# Autodesk Inventor assembly: drive with fourbar linkage
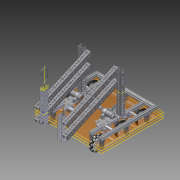
[picture p0: Inventor's stored thumbnail of the model, 180x180]
Saved by Autodesk Inventor 2013 (Build 170138000, 138)
## iProperties
Created: 2013-12-21
Part Number: drive with fourbar linkage
Document SubType Name: Assembly
Designer: kahohbein
Author: kahohbein
## Documents named in this file (12)
- C:\Users\kahohbein\Documents\GitHub\2013-2014_BlockParty\CAD\drive with fourbar linkage.iam
- C:\Users\kahohbein\Documents\GitHub\2013-2014_BlockParty\CAD\Drive\Final Drive Complete\Driveopen2.iam
- C:\Users\kahohbein\Documents\GitHub\2013-2014_BlockParty\CAD\COTSParts\Tetrix\Tetrix flat plate.ipt
- C:\Users\kahohbein\Documents\GitHub\2013-2014_BlockParty\CAD\COTSParts\Tetrix\Tetrix channel 288mm.ipt
- C:\Users\kahohbein\Documents\GitHub\2013-2014_BlockParty\CAD\COTSParts\Tetrix\Tetrix channel 32mm.ipt
- C:\Users\kahohbein\Documents\GitHub\2013-2014_BlockParty\CAD\COTSParts\Tetrix\Tetrix Channel 416mm.ipt
- C:\Users\kahohbein\Documents\GitHub\2013-2014_BlockParty\CAD\COTSParts\Tetrix\Bronze bushing.ipt
- C:\Users\kahohbein\Documents\GitHub\2013-2014_BlockParty\CAD\COTSParts\Tetrix\Tetrix channel 160mm.ipt
- C:\Users\kahohbein\Documents\GitHub\2013-2014_BlockParty\CAD\Tetrix channel 288mm modifyed.ipt
- C:\Users\kahohbein\Documents\GitHub\2013-2014_BlockParty\CAD\Lift\MK3\winch MK3.iam
- C:\Users\kahohbein\Documents\GitHub\2013-2014_BlockParty\CAD\COTSParts\Tetrix\Tetrix motor mount.ipt
- C:\Users\kahohbein\Documents\GitHub\2013-2014_BlockParty\CAD\Lift\MK3\hook prototype.ipt
## Components (29 placed, 11 different names)
1. Driveopen2:1 [sub-assembly] — Mate:1, Mate:2, Mate:3, Mate:4, Mate:5, Mate:6
2. Tetrix flat plate:1 — Mate:2, Mate:3, Mate:4, Mate:8, Mate:9, Mate:15, Mate:16, Mate:65, Mate:66, Mate:70
3. Tetrix flat plate:2 — Mate:1, Mate:5, Mate:6, Mate:7, Mate:10, Mate:11, Mate:12, Mate:67, Mate:68, Mate:69
4. Tetrix channel 288mm:1 — Mate:7, Mate:10, Mate:13, Mate:14, Mate:19, Mate:31, Mate:32, Mate:35, Mate:36, Mate:43, Mate:44, Mate:47, Mate:48
5. Tetrix channel 288mm:2 — Mate:8, Mate:9, Mate:17, Mate:18, Mate:20, Mate:25, Mate:28, Mate:29, Mate:30, Mate:38, Mate:41, Mate:42, Mate:50, Mate:51
6. Tetrix channel 32mm:1 — Mate:15, Mate:16, Mate:17, Mate:18
7. Tetrix channel 32mm:2 — Mate:11, Mate:12, Mate:13, Mate:14
8. Tetrix Channel 416mm:1 — Mate:20, Mate:21, Mate:24, Mate:26, Mate:74, Mate:75
9. Tetrix Channel 416mm:2 — Mate:19, Mate:21, Mate:33, Mate:34, Mate:60, Mate:61
10. Tetrix Channel 416mm:3 — Mate:38, Mate:39, Mate:40, Mate:53, Mate:55, Mate:59
11. Tetrix Channel 416mm:4 — Mate:39, Mate:45, Mate:46, Mate:55, Mate:73
12. Bronze bushing:1 — Mate:24, Mate:26, Mate:27
13. Bronze bushing:2 — Mate:25, Mate:27, Mate:28
14. Bronze bushing:3 — Mate:29, Mate:30
15. Bronze bushing:4 — Mate:31, Mate:36, Mate:37
16. Bronze bushing:5 — Mate:33, Mate:34, Mate:37
17. Bronze bushing:6 — Mate:32, Mate:35
18. Bronze bushing:7 — Mate:41, Mate:51
19. Bronze bushing:8 — Mate:42, Mate:50, Mate:52
20. Bronze bushing:9 — Mate:45, Mate:46, Mate:52
21. Bronze bushing:10 — Mate:40, Mate:53, Mate:54
22. Bronze bushing:11 — Mate:44, Mate:48, Mate:54
23. Bronze bushing:12 — Mate:43, Mate:47
24. Tetrix channel 288mm modifyed:1 — Mate:59, Mate:60, Mate:61, Mate:76, Mate:77, Mate:78
25. winch MK3:1 [sub-assembly] — Mate:71, Mate:72
26. Tetrix motor mount:1 — Mate:65, Mate:66, Mate:70, Mate:71
27. Tetrix motor mount:2 — Mate:67, Mate:68, Mate:69, Mate:72
28. Tetrix channel 160mm:1 — Mate:73, Mate:74, Mate:75
29. hook prototype:1 — Mate:76, Mate:77, Mate:78
## Relationships (69: Mate 69)
- Mate:1: Driveopen2:1 ↔ Tetrix flat plate:2
- Mate:2: Driveopen2:1 ↔ Tetrix flat plate:1
- Mate:3 (139.7 mm): Driveopen2:1 ↔ Tetrix flat plate:1
- Mate:4 (63.5 mm): Driveopen2:1 ↔ Tetrix flat plate:1
- Mate:5 (139.7 mm): Driveopen2:1 ↔ Tetrix flat plate:2
- Mate:6 (63.5 mm): Driveopen2:1 ↔ Tetrix flat plate:2
- Mate:7: Tetrix flat plate:2 ↔ Tetrix channel 288mm:1
- Mate:8: Tetrix flat plate:1 ↔ Tetrix channel 288mm:2
- Mate:9: Tetrix flat plate:1 ↔ Tetrix channel 288mm:2
- Mate:10: Tetrix flat plate:2 ↔ Tetrix channel 288mm:1
- Mate:11: Tetrix flat plate:2 ↔ Tetrix channel 32mm:2
- Mate:12: Tetrix flat plate:2 ↔ Tetrix channel 32mm:2
- Mate:13: Tetrix channel 288mm:1 ↔ Tetrix channel 32mm:2
- Mate:14: Tetrix channel 288mm:1 ↔ Tetrix channel 32mm:2
- Mate:15: Tetrix flat plate:1 ↔ Tetrix channel 32mm:1
- Mate:16: Tetrix flat plate:1 ↔ Tetrix channel 32mm:1
- Mate:17: Tetrix channel 288mm:2 ↔ Tetrix channel 32mm:1
- Mate:18: Tetrix channel 288mm:2 ↔ Tetrix channel 32mm:1
- Mate:19: Tetrix channel 288mm:1 ↔ Tetrix Channel 416mm:2
- Mate:20: Tetrix channel 288mm:2 ↔ Tetrix Channel 416mm:1
- Mate:21: Tetrix Channel 416mm:1 ↔ Tetrix Channel 416mm:2
- Mate:24: Tetrix Channel 416mm:1 ↔ Bronze bushing:1
- Mate:25: Tetrix channel 288mm:2 ↔ Bronze bushing:2
- Mate:26: Tetrix Channel 416mm:1 ↔ Bronze bushing:1
- Mate:27 (6.35 mm): Bronze bushing:1 ↔ Bronze bushing:2
- Mate:28: Tetrix channel 288mm:2 ↔ Bronze bushing:2
- Mate:29: Tetrix channel 288mm:2 ↔ Bronze bushing:3
- Mate:30: Tetrix channel 288mm:2 ↔ Bronze bushing:3
- Mate:31: Tetrix channel 288mm:1 ↔ Bronze bushing:4
- Mate:32: Tetrix channel 288mm:1 ↔ Bronze bushing:6
- Mate:33: Tetrix Channel 416mm:2 ↔ Bronze bushing:5
- Mate:34: Tetrix Channel 416mm:2 ↔ Bronze bushing:5
- Mate:35: Tetrix channel 288mm:1 ↔ Bronze bushing:6
- Mate:36: Tetrix channel 288mm:1 ↔ Bronze bushing:4
- Mate:37 (6.35 mm): Bronze bushing:4 ↔ Bronze bushing:5
- Mate:38: Tetrix channel 288mm:2 ↔ Tetrix Channel 416mm:3
- Mate:39: Tetrix Channel 416mm:3 ↔ Tetrix Channel 416mm:4
- Mate:40: Tetrix Channel 416mm:3 ↔ Bronze bushing:10
- Mate:41: Tetrix channel 288mm:2 ↔ Bronze bushing:7
- Mate:42: Tetrix channel 288mm:2 ↔ Bronze bushing:8
- Mate:43: Tetrix channel 288mm:1 ↔ Bronze bushing:12
- Mate:44: Tetrix channel 288mm:1 ↔ Bronze bushing:11
- Mate:45: Tetrix Channel 416mm:4 ↔ Bronze bushing:9
- Mate:46: Tetrix Channel 416mm:4 ↔ Bronze bushing:9
- Mate:47: Tetrix channel 288mm:1 ↔ Bronze bushing:12
- Mate:48: Tetrix channel 288mm:1 ↔ Bronze bushing:11
- Mate:50: Tetrix channel 288mm:2 ↔ Bronze bushing:8
- Mate:51: Tetrix channel 288mm:2 ↔ Bronze bushing:7
- Mate:52 (6.35 mm): Bronze bushing:8 ↔ Bronze bushing:9
- Mate:53: Tetrix Channel 416mm:3 ↔ Bronze bushing:10
- Mate:54 (6.35 mm): Bronze bushing:10 ↔ Bronze bushing:11
- Mate:55: Tetrix Channel 416mm:3 ↔ Tetrix Channel 416mm:4
- Mate:59: Tetrix Channel 416mm:3 ↔ Tetrix channel 288mm modifyed:1
- Mate:60: Tetrix Channel 416mm:2 ↔ Tetrix channel 288mm modifyed:1
- Mate:61 (3.175 mm): Tetrix Channel 416mm:2 ↔ Tetrix channel 288mm modifyed:1
- Mate:65: Tetrix flat plate:1 ↔ Tetrix motor mount:1
- Mate:66: Tetrix flat plate:1 ↔ Tetrix motor mount:1
- Mate:67: Tetrix flat plate:2 ↔ Tetrix motor mount:2
- Mate:68: Tetrix flat plate:2 ↔ Tetrix motor mount:2
- Mate:69: Tetrix flat plate:2 ↔ Tetrix motor mount:2
- Mate:70: Tetrix flat plate:1 ↔ Tetrix motor mount:1
- Mate:71: winch MK3:1 ↔ Tetrix motor mount:1
- Mate:72: winch MK3:1 ↔ Tetrix motor mount:2
- Mate:73: Tetrix Channel 416mm:4 ↔ Tetrix channel 160mm:1
- Mate:74: Tetrix Channel 416mm:1 ↔ Tetrix channel 160mm:1
- Mate:75 (3.175 mm): Tetrix Channel 416mm:1 ↔ Tetrix channel 160mm:1
- Mate:76: Tetrix channel 288mm modifyed:1 ↔ hook prototype:1
- Mate:77 (12.7 mm): Tetrix channel 288mm modifyed:1 ↔ hook prototype:1
- Mate:78 (12.7 mm): Tetrix channel 288mm modifyed:1 ↔ hook prototype:1
